# Autodesk Inventor assembly: TheDream
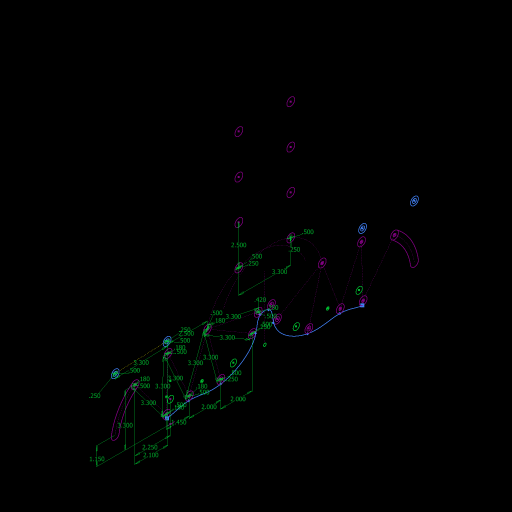
[picture p0: Inventor's stored thumbnail of the model, 512x512]
Saved by Autodesk Inventor 2024.1 (Build 281209000, 209)
## iProperties
Created: 2025-06-20
Part Number: TheDream
Document SubType Name: Assembly
Designer: Teddy
Author: Teddy
## Documents named in this file (7)
- C:\Users\Teddy\OneDrive\Desktop\VEX-CAD-Inventor-1.4.0\pushBack\PushBackBot2\InADreamBot\TheDream.iam
- C:\Users\Teddy\OneDrive\Desktop\VEX-CAD-Inventor-1.4.0\Motion\Wheels\Omni Wheel\2.75 Omni AS, Circle.iam
- C:\Users\Teddy\OneDrive\Desktop\VEX-CAD-Inventor-1.4.0\Motion\Wheels\Omni Wheel.iam
- C:\Users\Teddy\OneDrive\Desktop\VEX-CAD-Inventor-1.4.0\pushBack\PushBackBot2\InADreamBot\OuterDrive3DP.ipt
- C:\Users\Teddy\OneDrive\Desktop\VEX-CAD-Inventor-1.4.0\Structure\C Channel\Aluminum 1x2x1\Alu C 1x2x1x26.ipt
- C:\Users\Teddy\OneDrive\Desktop\VEX-CAD-Inventor-1.4.0\2024-25 VexGame\GearDriveTrain\WheelGear.ipt
- C:\Users\Teddy\OneDrive\Desktop\VEX-CAD-Inventor-1.4.0\pushBack\PushBackBot2\InADreamBot\IntakeMetal.ipt
## Components (11 placed, 5 different names)
1. OuterDrive3DP:1 — Insert:1, Insert:2, Insert:3, Insert:4
2. 2.75 Omni AS, Circle:1 [sub-assembly] — Insert:1, Insert:5, Insert:10
3. 2.75 Omni AS, Circle:2 [sub-assembly] — Insert:4, Insert:9
4. 2.75 Omni AS, Circle:3 [sub-assembly] — Insert:2, Insert:8
5. 2.75 Omni AS, Circle:4 [sub-assembly] — Insert:3, Insert:6, Insert:7
6. Alu C 1x2x1x26:1 — Insert:5, Insert:6
7. WheelGear:1 — Insert:7
8. WheelGear:2 — Insert:8
9. WheelGear:3 — Insert:9
10. WheelGear:4 — Insert:10, Flush:1, Flush:2
11. IntakeMetal:1 — Flush:1, Flush:2
## Relationships (12: Insert 10, Flush 2)
- Insert:1 (6.35 mm): OuterDrive3DP:1 ↔ 2.75 Omni AS, Circle:1
- Insert:2 (6.35 mm): OuterDrive3DP:1 ↔ 2.75 Omni AS, Circle:3
- Insert:3 (6.35 mm): OuterDrive3DP:1 ↔ 2.75 Omni AS, Circle:4
- Insert:4 (6.35 mm): OuterDrive3DP:1 ↔ 2.75 Omni AS, Circle:2
- Insert:5 (6.35 mm): 2.75 Omni AS, Circle:1 ↔ Alu C 1x2x1x26:1
- Insert:6 (6.35 mm): 2.75 Omni AS, Circle:4 ↔ Alu C 1x2x1x26:1
- Insert:7: 2.75 Omni AS, Circle:4 ↔ WheelGear:1
- Insert:8: 2.75 Omni AS, Circle:3 ↔ WheelGear:2
- Insert:9: 2.75 Omni AS, Circle:2 ↔ WheelGear:3
- Insert:10: 2.75 Omni AS, Circle:1 ↔ WheelGear:4
- Flush:1: WheelGear:4 ↔ IntakeMetal:1
- Flush:2: WheelGear:4 ↔ IntakeMetal:1
